# Autodesk Inventor assembly: Assembly1
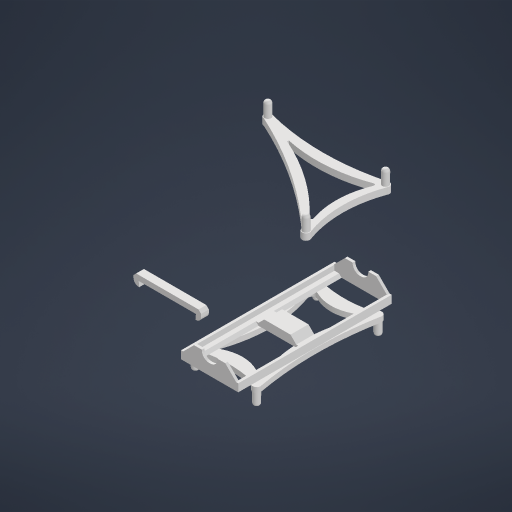
[picture p0: Inventor's stored thumbnail of the model, 512x512]
Saved by Autodesk Inventor 2024 (Build 280153000, 153)
## iProperties
Created: 2023-10-15
Part Number: Assembly1
Document SubType Name: Assembly
Designer: Gurra
Author: Gurra
## Documents named in this file (5)
- C:\Users\Gurra\Documents\GitRepos\MDU-SamarbetanderobotarDVA138\Projekt\CAD\Base\Assembly1.iam
- C:\Users\Gurra\Documents\GitRepos\MDU-SamarbetanderobotarDVA138\Projekt\CAD\Base\MotorHolder\BasePlate.ipt
- C:\Users\Gurra\Documents\GitRepos\MDU-SamarbetanderobotarDVA138\Projekt\CAD\Base\SiSpeedHolder\SiSpeedM1W_Holder.ipt
- C:\Users\Gurra\Documents\GitRepos\MDU-SamarbetanderobotarDVA138\Projekt\CAD\Hjul\Esp32_Holder.ipt
- C:\Users\Gurra\Documents\GitRepos\MDU-SamarbetanderobotarDVA138\Projekt\CAD\Base\Clip\Clip.ipt
## Components (4 placed, 4 different names)
1. BasePlate:1 — Mate:1
2. SiSpeedM1W_Holder:1
3. Esp32_Holder:1 — Mate:1
4. Clip:1
## Relationships (1: Mate 1)
- Mate:1: BasePlate:1 ↔ Esp32_Holder:1
